# Autodesk Inventor assembly: Segment_1
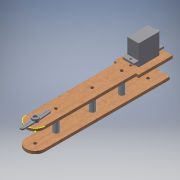
[picture p0: Inventor's stored thumbnail of the model, 180x180]
Saved by Autodesk Inventor 2017 (Build 210142000, 142)
## iProperties
Part Number: Segment_1
Material: Ogólny
Document SubType Name: Assembly
Designer: Damian
Author: Damian
## Documents named in this file (6)
- C:\Users\Damian\Documents\Inventor\Nowe\2.0\Segment_1.iam
- C:\Users\Damian\Documents\Inventor\Nowe\2.0\Część2.ipt
- C:\Users\Damian\Documents\Inventor\Nowe\2.0\Część1.ipt
- C:\Users\Damian\Documents\Inventor\Nowe\2.0\tuleja18.ipt
- C:\Users\Damian\Documents\Inventor\Nowe\2.0\towerpro.ipt
- C:\Users\Damian\Documents\Inventor\Nowe\2.0\Micro Servo 9g Arm.ipt
## Components (7 placed, 5 different names)
1. Część2:1 — Sztywne:1, Sztywne:5, Sztywne:7
2. Część1:1 — Sztywne:1, Sztywne:3, Sztywne:4, Sztywne:6
3. tuleja18:1 — Sztywne:6
4. tuleja18:2 — Sztywne:3
5. tuleja18:3 — Sztywne:4
6. towerpro:1 — Sztywne:5
7. Micro Servo 9g Arm:1 — Sztywne:7
## Relationships (6: WeldJoint 6)
- Sztywne:1 [WeldJoint] (18 mm): Część2:1 ↔ Część1:1
- Sztywne:3 [WeldJoint]: Część1:1 ↔ tuleja18:2
- Sztywne:4 [WeldJoint]: Część1:1 ↔ tuleja18:3
- Sztywne:5 [WeldJoint] (4 mm): Część2:1 ↔ towerpro:1
- Sztywne:6 [WeldJoint]: Część1:1 ↔ tuleja18:1
- Sztywne:7 [WeldJoint]: Część2:1 ↔ Micro Servo 9g Arm:1
